# Autodesk Inventor assembly: Задний_столб
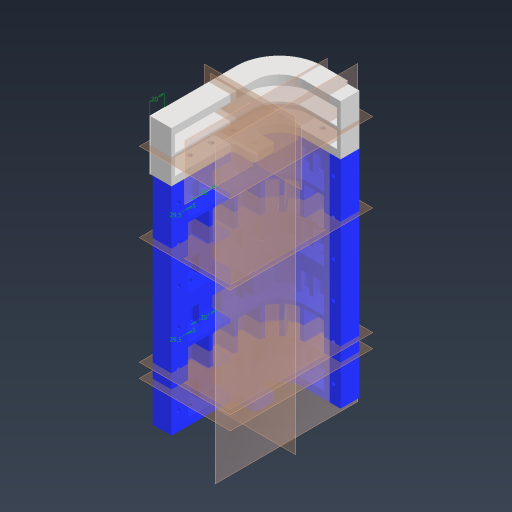
[picture p0: Inventor's stored thumbnail of the model, 512x512]
Saved by Autodesk Inventor 2023.2 (Build 272271030, 271C)
## iProperties
Created: 2025-09-30
Part Number: Задний_столб
Document SubType Name: Assembly
Designer: Олег Коноваленко
Author: Олег Коноваленко
## Documents named in this file (3)
- D:\!Rover\Rover\Rover_construction\Задний_столб.iam
- D:\!Rover\Rover\Rover_construction\Столб_версия_2.0.ipt
- D:\!Rover\Rover\Rover_construction\Верхняя часть столба зада.ipt
## Components (3 placed, 2 different names)
1. Столб_версия_2.0:1 — Совмещение:1, Заподлицо:1, Заподлицо:2
2. Столб_версия_2.0:2 — Совмещение:1, Заподлицо:1, Заподлицо:2, Совмещение:2, Заподлицо:3, Заподлицо:4
3. Верхняя часть столба зада:1 — Совмещение:2, Заподлицо:3, Заподлицо:4
## Relationships (6: Flush 4, Mate 2)
- Совмещение:1 [Mate]: Столб_версия_2.0:1 ↔ Столб_версия_2.0:2
- Заподлицо:1 [Flush]: Столб_версия_2.0:1 ↔ Столб_версия_2.0:2
- Заподлицо:2 [Flush]: Столб_версия_2.0:1 ↔ Столб_версия_2.0:2
- Совмещение:2 [Mate]: Столб_версия_2.0:2 ↔ Верхняя часть столба зада:1
- Заподлицо:3 [Flush]: Столб_версия_2.0:2 ↔ Верхняя часть столба зада:1
- Заподлицо:4 [Flush]: Столб_версия_2.0:2 ↔ Верхняя часть столба зада:1
